# Autodesk Inventor assembly: Assembly Latest
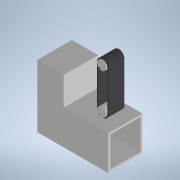
[picture p0: Inventor's stored thumbnail of the model, 180x180]
Saved by Autodesk Inventor 2022.2 (Build 262287000, 287)
## iProperties
Created: 2022-02-21
Part Number: Assembly Latest
Document SubType Name: Assembly
Designer: PRASHANTH
Author: PRASHANTH
## Documents named in this file (8)
- E:\BME\Autodesk Sample\Assembly Latest.iam
- E:\BME\Autodesk Sample\Part4.ipt
- E:\BME\Autodesk Sample\Part5.ipt
- E:\BME\Autodesk Sample\Part6.ipt
- E:\BME\Autodesk Sample\Part7.ipt
- E:\BME\Autodesk Sample\Part8.ipt
- E:\BME\Autodesk Sample\Part9.ipt
- E:\BME\Autodesk Sample\Assembly of Conveyor Belt.iam
## Components (9 placed, 7 different names)
1. Part4:1 — Mate:1, Flush:1, Flush:2, Flush:4, Flush:15
2. Part5:1 — Mate:1, Flush:1, Flush:2, Flush:3, Mate:2, Flush:5, Mate:3, Flush:6
3. Part6:1 — Flush:3, Mate:2, Flush:4, Mate:4, Flush:7, Flush:8
4. Part6:2 — Flush:5, Mate:3, Flush:6, Flush:9, Flush:10, Mate:5
5. Part7:1 — Flush:9, Flush:10, Mate:5, Mate:6, Flush:11, Flush:14, Flush:16
6. Part7:2 — Mate:4, Flush:7, Flush:8, Flush:12, Flush:13, Mate:7
7. Part8:1 — Mate:6, Flush:11, Flush:12
8. Part9:1 — Flush:13, Mate:7, Flush:14, Mate:8
9. Assembly of Conveyor Belt:1 [sub-assembly] — Flush:15, Flush:16, Mate:8
## Relationships (24: Flush 16, Mate 8)
- Mate:1: Part4:1 ↔ Part5:1
- Flush:1: Part4:1 ↔ Part5:1
- Flush:2: Part4:1 ↔ Part5:1
- Flush:3: Part5:1 ↔ Part6:1
- Mate:2: Part5:1 ↔ Part6:1
- Flush:4: Part4:1 ↔ Part6:1
- Flush:5: Part5:1 ↔ Part6:2
- Mate:3: Part5:1 ↔ Part6:2
- Flush:6: Part5:1 ↔ Part6:2
- Mate:4: Part6:1 ↔ Part7:2
- Flush:7: Part6:1 ↔ Part7:2
- Flush:8: Part6:1 ↔ Part7:2
- Flush:9: Part6:2 ↔ Part7:1
- Flush:10: Part6:2 ↔ Part7:1
- Mate:5: Part6:2 ↔ Part7:1
- Mate:6: Part7:1 ↔ Part8:1
- Flush:11: Part7:1 ↔ Part8:1
- Flush:12: Part7:2 ↔ Part8:1
- Flush:13: Part7:2 ↔ Part9:1
- Mate:7: Part7:2 ↔ Part9:1
- Flush:14: Part7:1 ↔ Part9:1
- Flush:15 (-190 mm): Part4:1 ↔ Assembly of Conveyor Belt:1
- Flush:16 (60 mm): Part7:1 ↔ Assembly of Conveyor Belt:1
- Mate:8 (50 mm): Part9:1 ↔ Assembly of Conveyor Belt:1
